# Autodesk Inventor assembly: Intake motor on xrail left
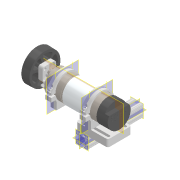
[picture p0: Inventor's stored thumbnail of the model, 180x180]
Saved by Autodesk Inventor 2020 (Build 240168000, 168)
## iProperties
Created: 2020-01-13
Part Number: Intake motor on xrail left
Document SubType Name: Assembly
Designer: ball
Author: ball
## Documents named in this file (5)
- C:\FTC\FTC8863CAD\2019 Robot\Collection\Intake motor on xrail left.iam
- C:\FTC\FTC8863CAD\2019 Robot\Collection\neverest 40 + mounts.iam
- C:\FTC\FTC8863CAD\2019 Robot\Collection\compliant wheel 2 in + 6mm shaft adapterr.iam
- C:\FTC\FTC8863CAD\Actobotics\565 parts\xrail_3.5in.ipt
- C:\FTC\FTC8863CAD\2019 Robot\Collection\intake motor mount to xrail.ipt
## Components (4 placed, 4 different names)
1. neverest 40 + mounts:1 [sub-assembly]
2. compliant wheel 2 in + 6mm shaft adapterr:1 [sub-assembly]
3. xrail_3.5in:1
4. intake motor mount to xrail:1
## Relationships (6: Mate 4, Flush 2)
- [Mate]: neverest 40 + mounts:1 ↔ compliant wheel 2 in + 6mm shaft adapterr:1
- [Mate]: neverest 40 + mounts:1 ↔ compliant wheel 2 in + 6mm shaft adapterr:1
- [Mate]: xrail_3.5in:1 ↔ intake motor mount to xrail:1
- [Flush]: xrail_3.5in:1 ↔ intake motor mount to xrail:1
- [Flush]: xrail_3.5in:1 ↔ intake motor mount to xrail:1
- [Mate]: neverest 40 + mounts:1 ↔ intake motor mount to xrail:1
